# Autodesk Inventor assembly: Drive Wheel Assembly V2
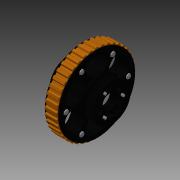
[picture p0: Inventor's stored thumbnail of the model, 180x180]
Saved by Autodesk Inventor 2013 (Build 170138000, 138)
## iProperties
Created: 2013-01-17
Part Number: Drive Wheel Assembly V2
Document SubType Name: Assembly
Designer: Moses
Mass: 519.978 g
Surface Area: 1902.31 cm^2
Volume: 424.399 cm^3
Density: 1.22521 g/cm^3
Author: Moses
## Documents named in this file (5)
- C:\Users\Moses\Documents\GitHub\frc2013CAD\Drivetrain\Drive Wheel Assembly V2.iam
- C:\Users\Moses\Documents\GitHub\frc2013CAD\Drivetrain\6Plaction-asm\6Plaction-asm.iam
- C:\Users\Moses\Documents\GitHub\frc2013CAD\Drivetrain\Custom Belt Pulley Hex Hub.ipt
- C:\Users\Moses\Documents\GitHub\frc2013CAD\Drivetrain\DBK_42ToothPulley (am-2234)\DBK_42ToothPulley V2.iam
- C:\Users\Moses\Documents\GitHub\frc2013CAD\Drivetrain\91251A980 10-24 Screw\91251A980.ipt
## Components (8 placed, 4 different names)
1. 6Plaction-asm:1 [sub-assembly] — Mate:1, Mate:2, Mate:3, Mate:4, Mate:5, Mate:6
2. Custom Belt Pulley Hex Hub:1 — Mate:1, Mate:2, Mate:3, Mate:10, Mate:11, Mate:12
3. Custom Belt Pulley Hex Hub:2 — Mate:4, Mate:5, Mate:6, Mate:7, Mate:8, Mate:9
4. DBK_42ToothPulley V2:1 [sub-assembly] — Mate:7, Mate:8, Mate:9, Insert:1, Insert:2, Insert:3
5. DBK_42ToothPulley V2:2 [sub-assembly] — Mate:10, Mate:11, Mate:12
6. 91251A980:1 — Insert:1
7. 91251A980:2 — Insert:2
8. 91251A980:3 — Insert:3
## Relationships (15: Mate 12, Insert 3)
- Mate:1: 6Plaction-asm:1 ↔ Custom Belt Pulley Hex Hub:1
- Mate:2: 6Plaction-asm:1 ↔ Custom Belt Pulley Hex Hub:1
- Mate:3: 6Plaction-asm:1 ↔ Custom Belt Pulley Hex Hub:1
- Mate:4: 6Plaction-asm:1 ↔ Custom Belt Pulley Hex Hub:2
- Mate:5: 6Plaction-asm:1 ↔ Custom Belt Pulley Hex Hub:2
- Mate:6: 6Plaction-asm:1 ↔ Custom Belt Pulley Hex Hub:2
- Mate:7: Custom Belt Pulley Hex Hub:2 ↔ DBK_42ToothPulley V2:1
- Mate:8: Custom Belt Pulley Hex Hub:2 ↔ DBK_42ToothPulley V2:1
- Mate:9: Custom Belt Pulley Hex Hub:2 ↔ DBK_42ToothPulley V2:1
- Mate:10: Custom Belt Pulley Hex Hub:1 ↔ DBK_42ToothPulley V2:2
- Mate:11: Custom Belt Pulley Hex Hub:1 ↔ DBK_42ToothPulley V2:2
- Mate:12: Custom Belt Pulley Hex Hub:1 ↔ DBK_42ToothPulley V2:2
- Insert:1: DBK_42ToothPulley V2:1 ↔ 91251A980:1
- Insert:2: DBK_42ToothPulley V2:1 ↔ 91251A980:2
- Insert:3: DBK_42ToothPulley V2:1 ↔ 91251A980:3
